# Autodesk Inventor assembly: astacompleta301
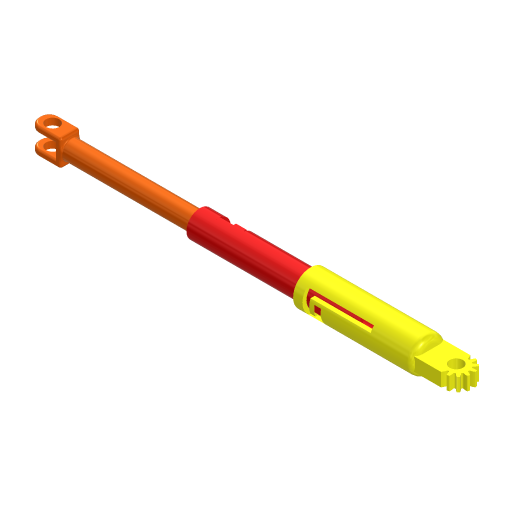
[picture p0: Inventor's stored thumbnail of the model, 512x512]
Saved by Autodesk Inventor 2024 (Build 280153000, 153)
## iProperties
Created: 2024-05-31
Part Number: astacompleta301
Document SubType Name: Assembly
Designer: alexz
Author: alexz
## Documents named in this file (4)
- C:\Users\alexz\Documents\Inventor\Esercizi\Progetto\astacompleta301.iam
- C:\Users\alexz\Documents\Inventor\Esercizi\Progetto\astaoscilla2_(310).ipt
- C:\Users\alexz\Documents\Inventor\Esercizi\Progetto\astaoscilla3_(301).ipt
- C:\Users\alexz\Documents\Inventor\Esercizi\Progetto\asteoscila1_(301).ipt
## Components (3 placed, 3 different names)
1. astaoscilla2_(310):1 — Cylindrical:1, Cylindrical:2
2. astaoscilla3_(301):1 — Cylindrical:2
3. asteoscila1_(301):1 — Cylindrical:1
## Relationships (2: CylindricalJoint 2)
- Cylindrical:1: astaoscilla2_(310):1 ↔ asteoscila1_(301):1
- Cylindrical:2: astaoscilla2_(310):1 ↔ astaoscilla3_(301):1
